# Autodesk Inventor assembly: LegChainTensioner
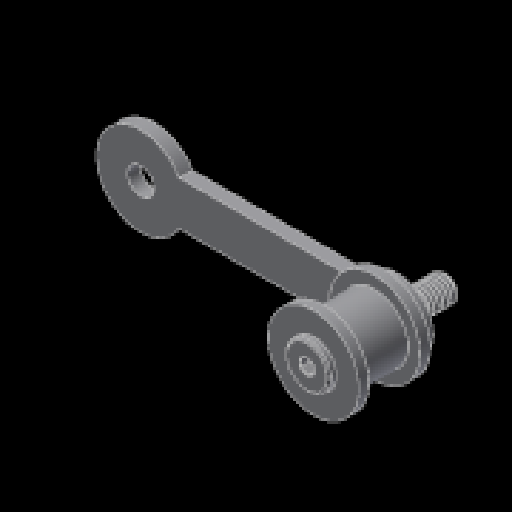
[picture p0: Inventor's stored thumbnail of the model, 512x512]
Saved by Autodesk Inventor 2025.2 (Build 292293000, 293)
## iProperties
Created: 2026-01-19
Part Number: LegChainTensioner
Document SubType Name: Assembly
Designer: valer
Author: valer
## Documents named in this file (4)
- C:\Users\valer\Desktop\str1ker\cad\LegChainTensioner.iam
- C:\Users\valer\Desktop\str1ker\cad\LegChainTensionerBlock.ipt
- C:\Users\valer\Desktop\str1ker\cad\external\91273A407_Same-Size Thread 18-8 Stainless Steel Shoulder Screw.ipt
- C:\Users\valer\Desktop\str1ker\cad\LegChainTensionerArm.ipt
## Components (3 placed, 3 different names)
1. LegChainTensionerBlock:1 — Mate:1, Mate:2, Mate:4
2. 91273A407_Same-Size Thread 18-8 Stainless Steel Shoulder Screw:1 — Mate:1, Mate:2, Mate:3
3. LegChainTensionerArm:1 — Mate:3, Mate:4
## Relationships (4: Mate 4)
- Mate:1: LegChainTensionerBlock:1 ↔ 91273A407_Same-Size Thread 18-8 Stainless Steel Shoulder Screw:1
- Mate:2: LegChainTensionerBlock:1 ↔ 91273A407_Same-Size Thread 18-8 Stainless Steel Shoulder Screw:1
- Mate:3: 91273A407_Same-Size Thread 18-8 Stainless Steel Shoulder Screw:1 ↔ LegChainTensionerArm:1
- Mate:4: LegChainTensionerBlock:1 ↔ LegChainTensionerArm:1
